# Autodesk Inventor assembly: GE-12102
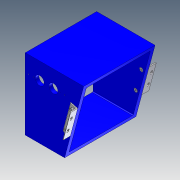
[picture p0: Inventor's stored thumbnail of the model, 180x180]
Saved by Autodesk Inventor 2012 (Build 160160000, 160)
## iProperties
Created: 2011-10-29
Part Number: GE-12102
Document SubType Name: Assembly
Designer: dfoster
Description: Sensor Box Assembly
Title: Sensor Box Assembly
Author: dfoster
## Documents named in this file (5)
- C:\Data Folder\FRC 2012 Field\Components\GE-12102.iam
- C:\Data Folder\FRC 2012 Field\Components\GE-12059.ipt
- C:\Data Folder\FRC 2012 Field\Components\GE-12054.ipt
- C:\Data Folder\FRC 2012 Field\Components\HW-00074.ipt
- C:\Data Folder\FRC 2012 Field\Components\HW-00002.ipt
## Components (11 placed, 4 different names)
1. GE-12059:1 — Mate:1, Mate:2, Mate:3, Mate:4, Mate:5, Mate:6, Flush:1, Mate:7, Flush:2, Mate:8
2. GE-12054:1 — Mate:1, Mate:2, Mate:3, Insert:1
3. GE-12054:2 — Mate:4, Mate:5, Mate:6, Insert:2
4. HW-00074:1 — Flush:2, Mate:8
5. HW-00074:2 — Flush:1, Mate:7
6. HW-00002:1 — Insert:1
7. HW-00002:2 — Insert:2
8. HW-00074:3
9. HW-00074:4
10. HW-00002:3
11. HW-00002:4
## Component patterns: (2 elements, first: HW-00074:1 + HW-00074:2 + HW-00002:1 + HW-00002:2)
## Relationships (12: Mate 8, Flush 2, Insert 2)
- Mate:1: GE-12059:1 ↔ GE-12054:1
- Mate:2: GE-12059:1 ↔ GE-12054:1
- Mate:3: GE-12059:1 ↔ GE-12054:1
- Mate:4: GE-12059:1 ↔ GE-12054:2
- Mate:5: GE-12059:1 ↔ GE-12054:2
- Mate:6: GE-12059:1 ↔ GE-12054:2
- Flush:1: GE-12059:1 ↔ HW-00074:2
- Mate:7: GE-12059:1 ↔ HW-00074:2
- Flush:2: GE-12059:1 ↔ HW-00074:1
- Mate:8: GE-12059:1 ↔ HW-00074:1
- Insert:1: GE-12054:1 ↔ HW-00002:1
- Insert:2: GE-12054:2 ↔ HW-00002:2
